# Autodesk Inventor assembly: Box Assembly
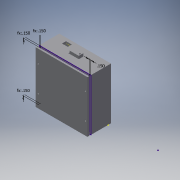
[picture p0: Inventor's stored thumbnail of the model, 180x180]
Saved by Autodesk Inventor 2018 (Build 220112000, 112)
## iProperties
Created: 2018-04-20
Part Number: Box Assembly
Document SubType Name: Assembly
Designer: MIABo
Author: MIABo
## Documents named in this file (3)
- C:\Users\MIABo\Documents\GitHub\Robotics_Challenge_Beacon\Box Assembly.iam
- C:\Users\MIABo\Documents\GitHub\Robotics_Challenge_Beacon\Boxv2.ipt
- C:\Users\MIABo\Documents\GitHub\Robotics_Challenge_Beacon\Lid.ipt
## Components (2 placed, 2 different names)
1. Boxv2:1 — Insert:1, Insert:2
2. Lid:1 — Insert:1, Insert:2
## Relationships (2: Insert 2)
- Insert:1: Boxv2:1 ↔ Lid:1
- Insert:2: Boxv2:1 ↔ Lid:1
